# Autodesk Inventor assembly: spacerFinal
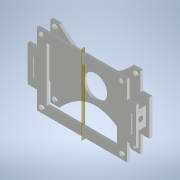
[picture p0: Inventor's stored thumbnail of the model, 180x180]
Saved by Autodesk Inventor 2020 (Build 240168000, 168)
## iProperties
Created: 2019-06-18
Part Number: spacerFinal
Document SubType Name: Assembly
Designer: Vivek Muskan
Author: Vivek Muskan
## Documents named in this file (4)
- C:\Users\Vivek Muskan\Documents\TARGET25\spacerFinal.iam
- C:\Users\Vivek Muskan\Documents\TARGET25\bottomBearingHolder.ipt
- C:\Users\Vivek Muskan\Documents\TARGET25\topBearingHolder.ipt
- C:\Users\Vivek Muskan\Documents\TARGET25\beringKundi.ipt
## Components (4 placed, 3 different names)
1. bottomBearingHolder:1 — Flush:1, Flush:2, Flush:3, Flush:7, Mate:3, Mate:4
2. topBearingHolder:1 — Flush:1, Flush:2, Flush:3, Mate:1, Mate:2, Flush:4
3. beringKundi:1 — Mate:1, Mate:2, Flush:4
4. beringKundi:2 — Flush:7, Mate:3, Mate:4
## Relationships (9: Flush 5, Mate 4)
- Flush:1 (7.5 mm): bottomBearingHolder:1 ↔ topBearingHolder:1
- Flush:2: bottomBearingHolder:1 ↔ topBearingHolder:1
- Flush:3: bottomBearingHolder:1 ↔ topBearingHolder:1
- Mate:1: topBearingHolder:1 ↔ beringKundi:1
- Mate:2: topBearingHolder:1 ↔ beringKundi:1
- Flush:4 (-0.5 mm): topBearingHolder:1 ↔ beringKundi:1
- Flush:7 (0.5 mm): bottomBearingHolder:1 ↔ beringKundi:2
- Mate:3: bottomBearingHolder:1 ↔ beringKundi:2
- Mate:4: bottomBearingHolder:1 ↔ beringKundi:2
